# Autodesk Inventor assembly: numbar-print
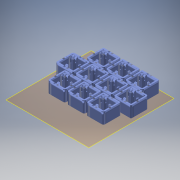
[picture p0: Inventor's stored thumbnail of the model, 180x180]
Saved by Autodesk Inventor 2018 (Build 220112000, 112)
## iProperties
Created: 2017-07-27
Part Number: numbar-print
Document SubType Name: Assembly
Designer: Jason Cemra
Author: Jason Cemra
## Documents named in this file (3)
- C:\Users\Jason Cemra\Documents\Logical Store\StenoToppers\stenotoppers\cherrymx\print-assemblies\numbar-print.iam
- C:\Users\Jason Cemra\Documents\Logical Store\StenoToppers\stenotoppers\cherrymx\stenotoppers\numbar_cmx.ipt
- C:\Users\Jason Cemra\Documents\Logical Store\StenoToppers\stenotoppers\cherrymx\stenotoppers.ipt
## Components (10 placed, 1 different names)
1. numbar_cmx:1 — Mate:1
2. numbar_cmx:2 — Mate:3
3. numbar_cmx:3
4. numbar_cmx:4
5. numbar_cmx:5
6. numbar_cmx:6
7. numbar_cmx:7 — Mate:2, Mate:3
8. numbar_cmx:8
9. numbar_cmx:9
10. numbar_cmx:10
## Component patterns: (6 elements, first: numbar_cmx:1), (4 elements, first: numbar_cmx:7)
## Relationships (3: Mate 3)
- Mate:1: numbar_cmx:1
- Mate:2: numbar_cmx:7
- Mate:3: numbar_cmx:2 ↔ numbar_cmx:7
